# Autodesk Inventor assembly: Assembly1
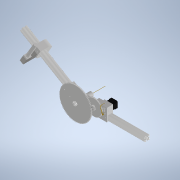
[picture p0: Inventor's stored thumbnail of the model, 180x180]
Saved by Autodesk Inventor 2022.3 (Build 263350000, 350)
## iProperties
Created: 2022-01-28
Part Number: Assembly1
Document SubType Name: Assembly
Designer: Martijn
Author: Martijn
## Documents named in this file (19)
- D:\phd\git\1dofsetup\Assembly1.iam
- D:\phd\git\1dofsetup\30x30x50.ipt
- D:\phd\git\1dofsetup\NEMA 17.ipt
- D:\phd\git\1dofsetup\pololu-universal-aluminum-mounting-hub-for-5mm-shaft-m3-holes.ipt
- D:\phd\git\1dofsetup\pololu-universal-aluminum-mounting-hub-for-8mm-shaft-m3-holes.ipt
- D:\phd\git\1dofsetup\SKF_608-2ZZ.ipt
- D:\phd\git\1dofsetup\load_cell.ipt
- D:\phd\git\1dofsetup\fixation_circle.ipt
- D:\phd\git\1dofsetup\8mm_to 6.35mm_kaplin.ipt
- D:\phd\git\1dofsetup\axis1.ipt
- D:\phd\git\1dofsetup\Lock Collar 8mm.ipt
- D:\phd\git\1dofsetup\axis2.ipt
- D:\phd\git\1dofsetup\handle_vertical.ipt
- D:\phd\git\1dofsetup\double_gear.ipt
- D:\phd\git\1dofsetup\nema_mount.ipt
- D:\phd\git\1dofsetup\double_gear_mount.ipt
- D:\phd\git\1dofsetup\loacell_mount2.ipt
- D:\phd\git\1dofsetup\bearing_mount_combined.ipt
- D:\phd\git\1dofsetup\big_gear_reinforced.ipt
## Components (24 placed, 18 different names)
1. 30x30x50:1 — Mate:188, Mate:189, Flush:50, Mate:201, Mate:202, Flush:51, Mate:205
2. 30x30x50:2 — Mate:168, Mate:169, Mate:175, Mate:176, Mate:192, Mate:193, Mate:196
3. NEMA 17:1 — Mate:143, Mate:170, Mate:171, Mate:172, Mate:182
4. pololu-universal-aluminum-mounting-hub-for-5mm-shaft-m3-holes:1 — Mate:143, Mate:144, Mate:145, Mate:182, Mate:183
5. pololu-universal-aluminum-mounting-hub-for-8mm-shaft-m3-holes:1 — Flush:43, Mate:159, Mate:207, Mate:208
6. SKF_608-2ZZ:2 — Mate:136, Mate:179
7. SKF_608-2ZZ:4 — Mate:157, Mate:200, Mate:203
8. load_cell:1 — Mate:160, Mate:161, Flush:49, Mate:190, Mate:191, Mate:206
9. fixation_circle:1 — Mate:144, Mate:145, Mate:183
10. 8mm_to 6.35mm_kaplin:1 — Mate:199
11. axis1:1 — Mate:77, Flush:30, Mate:136, Mate:174, Mate:184
12. Lock Collar 8mm:2 — Mate:77, Flush:30, Mate:178
13. SKF_608-2ZZ:5
14. axis2:1 — Flush:43, Mate:140, Mate:157, Mate:159, Mate:194, Mate:199, Mate:204, Mate:209
15. handle_vertical:1 — Mate:160, Mate:161, Flush:49
16. double_gear:1 — Mate:174, Mate:177, Mate:185
17. nema_mount:1 — Mate:168, Mate:169, Mate:170, Mate:171, Mate:172
18. double_gear_mount:1 — Mate:175, Mate:176, Mate:177, Mate:178, Mate:179, Mate:180, Mate:181
19. SKF_608-2ZZ:6 — Mate:180, Mate:181
20. Lock Collar 8mm:3 — Mate:184, Mate:185
21. loacell_mount2:1 — Mate:188, Mate:189, Flush:50, Mate:190, Mate:191, Mate:206
22. bearing_mount_combined:1 — Mate:192, Mate:193, Mate:194, Mate:196, Mate:200, Mate:210
23. big_gear_reinforced:2 — Mate:201, Mate:202, Mate:203, Mate:204, Flush:51, Mate:205, Mate:207, Mate:208
24. Lock Collar 8mm:4 — Mate:209, Mate:210
## Relationships (52: Mate 47, Flush 5)
- Mate:77: axis1:1 ↔ Lock Collar 8mm:2
- Flush:30 (0.5 mm): axis1:1 ↔ Lock Collar 8mm:2
- Flush:43: pololu-universal-aluminum-mounting-hub-for-8mm-shaft-m3-holes:1 ↔ axis2:1
- Mate:136: SKF_608-2ZZ:2 ↔ axis1:1
- Mate:140: axis2:1
- Mate:143: NEMA 17:1 ↔ pololu-universal-aluminum-mounting-hub-for-5mm-shaft-m3-holes:1
- Mate:144: pololu-universal-aluminum-mounting-hub-for-5mm-shaft-m3-holes:1 ↔ fixation_circle:1
- Mate:145: pololu-universal-aluminum-mounting-hub-for-5mm-shaft-m3-holes:1 ↔ fixation_circle:1
- Mate:157: SKF_608-2ZZ:4 ↔ axis2:1
- Mate:159: pololu-universal-aluminum-mounting-hub-for-8mm-shaft-m3-holes:1 ↔ axis2:1
- Mate:160: load_cell:1 ↔ handle_vertical:1
- Mate:161: load_cell:1 ↔ handle_vertical:1
- Flush:49: load_cell:1 ↔ handle_vertical:1
- Mate:168: 30x30x50:2 ↔ nema_mount:1
- Mate:169: 30x30x50:2 ↔ nema_mount:1
- Mate:170: NEMA 17:1 ↔ nema_mount:1
- Mate:171: NEMA 17:1 ↔ nema_mount:1
- Mate:172: NEMA 17:1 ↔ nema_mount:1
- Mate:174: axis1:1 ↔ double_gear:1
- Mate:175: 30x30x50:2 ↔ double_gear_mount:1
- Mate:176: 30x30x50:2 ↔ double_gear_mount:1
- Mate:177: double_gear:1 ↔ double_gear_mount:1
- Mate:178: Lock Collar 8mm:2 ↔ double_gear_mount:1
- Mate:179: SKF_608-2ZZ:2 ↔ double_gear_mount:1
- Mate:180: double_gear_mount:1 ↔ SKF_608-2ZZ:6
- Mate:181: double_gear_mount:1 ↔ SKF_608-2ZZ:6
- Mate:182 (6.5 mm): NEMA 17:1 ↔ pololu-universal-aluminum-mounting-hub-for-5mm-shaft-m3-holes:1
- Mate:183: pololu-universal-aluminum-mounting-hub-for-5mm-shaft-m3-holes:1 ↔ fixation_circle:1
- Mate:184: axis1:1 ↔ Lock Collar 8mm:3
- Mate:185: double_gear:1 ↔ Lock Collar 8mm:3
- Mate:188 (0.2 mm): 30x30x50:1 ↔ loacell_mount2:1
- Mate:189 (0.2 mm): 30x30x50:1 ↔ loacell_mount2:1
- Flush:50 (-100 mm): 30x30x50:1 ↔ loacell_mount2:1
- Mate:190: load_cell:1 ↔ loacell_mount2:1
- Mate:191: load_cell:1 ↔ loacell_mount2:1
- Mate:192 (0.2 mm): 30x30x50:2 ↔ bearing_mount_combined:1
- Mate:193 (0.2 mm): 30x30x50:2 ↔ bearing_mount_combined:1
- Mate:194: axis2:1 ↔ bearing_mount_combined:1
- Mate:196: 30x30x50:2 ↔ bearing_mount_combined:1
- Mate:199: 8mm_to 6.35mm_kaplin:1 ↔ axis2:1
- Mate:200: SKF_608-2ZZ:4 ↔ bearing_mount_combined:1
- Mate:201: 30x30x50:1 ↔ big_gear_reinforced:2
- Mate:202: 30x30x50:1 ↔ big_gear_reinforced:2
- Mate:203 (1 mm): SKF_608-2ZZ:4 ↔ big_gear_reinforced:2
- Mate:204: axis2:1 ↔ big_gear_reinforced:2
- Flush:51: 30x30x50:1 ↔ big_gear_reinforced:2
- Mate:205: 30x30x50:1 ↔ big_gear_reinforced:2
- Mate:206: load_cell:1 ↔ loacell_mount2:1
- Mate:207: pololu-universal-aluminum-mounting-hub-for-8mm-shaft-m3-holes:1 ↔ big_gear_reinforced:2
- Mate:208: pololu-universal-aluminum-mounting-hub-for-8mm-shaft-m3-holes:1 ↔ big_gear_reinforced:2
- Mate:209: axis2:1 ↔ Lock Collar 8mm:4
- Mate:210 (0.5 mm): bearing_mount_combined:1 ↔ Lock Collar 8mm:4
